# Autodesk Inventor assembly: Motor
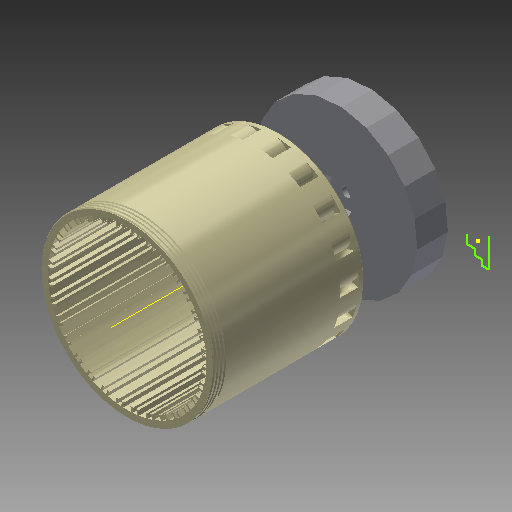
[picture p0: Inventor's stored thumbnail of the model, 512x512]
Saved by Autodesk Inventor 2017 (Build 210142000, 142)
## iProperties
Created: 2017-08-04
Part Number: Motor
Document SubType Name: Assembly
Designer: vmiguel
Mass: 7960.64 g
Surface Area: 19074.8 cm^2
Volume: 6750.82 cm^3
Density: 1.17921 g/cm^3
Author: vmiguel
## Documents named in this file (4)
- C:\Users\vmiguel\Dropbox\CarPlane\Motor\Motor.iam
- C:\Users\vmiguel\Dropbox\CarPlane\Motor\Rotor.ipt
- C:\Users\vmiguel\Dropbox\CarPlane\Motor\Blade.ipt
- C:\Users\vmiguel\Dropbox\CarPlane\Motor\PropellerHub.ipt
## Components (3 placed, 3 different names)
1. Rotor:1 — Mate:1
2. Blade:1
3. PropellerHub:1 — Mate:1
## Relationships (1: Mate 1)
- Mate:1: Rotor:1 ↔ PropellerHub:1
